# Autodesk Inventor assembly: Gantry Table With Chucks
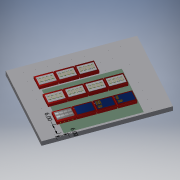
[picture p0: Inventor's stored thumbnail of the model, 180x180]
Saved by Autodesk Inventor 2019.4 (Build 234330000, 330)
## iProperties
Created: 2021-01-12
Part Number: Gantry Table With Chucks
Document SubType Name: Assembly
Designer: caleb
Author: caleb
## Documents named in this file (8)
- C:\Users\cfang\Desktop\nebraska-silicon-lab\Hardware\ETL\Module Assembly\Gantry Table With Chucks.iam
- C:\Users\cfang\Desktop\nebraska-silicon-lab\Hardware\ETL\Module Assembly\Gantry Base.ipt
- C:\Users\cfang\Desktop\nebraska-silicon-lab\Hardware\ETL\Module Assembly\Chuck with Assembly Plate.iam
- C:\Users\cfang\Desktop\nebraska-silicon-lab\Hardware\ETL\Module Assembly\Chuck with BBM Staging Plate.iam
- C:\Users\cfang\Desktop\nebraska-silicon-lab\Hardware\ETL\Module Assembly\Chuck with Glue Reservoir Plate.iam
- C:\Users\cfang\Desktop\nebraska-silicon-lab\Hardware\ETL\Module Assembly\Chuck with Glue Stamp Staging Plate.iam
- C:\Users\cfang\Desktop\nebraska-silicon-lab\Hardware\ETL\Module Assembly\Chuck\Chuck Assembly.iam
- C:\Users\cfang\Desktop\nebraska-silicon-lab\Hardware\ETL\Module Assembly\Glue Stamp Staging Plate\Assembly with Weights.iam
## Components (13 placed, 7 different names)
1. Gantry Base:1 — Mate:1, Mate:2, Mate:3, Mate:4, Angle:1, Angle:2, Angle:3, Angle:4, Mate:5, Angle:5, Mate:7, Mate:8, Mate:9, Angle:6, Angle:7, Angle:8, Mate:10, Mate:11, Mate:12, Angle:9, Angle:10, Angle:11, Insert:1, Insert:2, Insert:3, Insert:4, Insert:5, Insert:6, Insert:7, Insert:8, Insert:9, Insert:10, Insert:11
2. Chuck with Assembly Plate:1 [sub-assembly] — Mate:1, Angle:1, Insert:5
3. Chuck with BBM Staging Plate:1 [sub-assembly] — Mate:2, Angle:2, Insert:1
4. Chuck with Glue Reservoir Plate:1 [sub-assembly] — Mate:3, Angle:3, Insert:2
5. Chuck with Glue Stamp Staging Plate:1 [sub-assembly] — Mate:4, Angle:4, Insert:4
6. Chuck Assembly:1 [sub-assembly] — Mate:5, Angle:5, Mate:6, Tangent:1, Tangent:2, Tangent:3, Insert:3
7. Assembly with Weights:1 [sub-assembly] — Mate:6, Tangent:1, Tangent:2, Tangent:3
8. Chuck with Assembly Plate:2 [sub-assembly] — Mate:7, Angle:7, Insert:6
9. Chuck with Assembly Plate:3 [sub-assembly] — Mate:8, Angle:6, Insert:7
10. Chuck with Assembly Plate:4 [sub-assembly] — Mate:9, Angle:8, Insert:8
11. Chuck with Assembly Plate:5 [sub-assembly] — Mate:10, Angle:10, Insert:9
12. Chuck with Assembly Plate:6 [sub-assembly] — Mate:11, Angle:11, Insert:11
13. Chuck with Assembly Plate:7 [sub-assembly] — Mate:12, Angle:9, Insert:10
## Relationships (37: Mate 12, Angle 11, Insert 11, Tangent 3)
- Mate:1: Gantry Base:1 ↔ Chuck with Assembly Plate:1
- Mate:2: Gantry Base:1 ↔ Chuck with BBM Staging Plate:1
- Mate:3: Gantry Base:1 ↔ Chuck with Glue Reservoir Plate:1
- Mate:4: Gantry Base:1 ↔ Chuck with Glue Stamp Staging Plate:1
- Angle:1 (0 deg): Gantry Base:1 ↔ Chuck with Assembly Plate:1
- Angle:2 (0 deg): Gantry Base:1 ↔ Chuck with BBM Staging Plate:1
- Angle:3 (0 deg): Gantry Base:1 ↔ Chuck with Glue Reservoir Plate:1
- Angle:4 (0 deg): Gantry Base:1 ↔ Chuck with Glue Stamp Staging Plate:1
- Mate:5: Gantry Base:1 ↔ Chuck Assembly:1
- Angle:5 (0 deg): Gantry Base:1 ↔ Chuck Assembly:1
- Mate:6: Chuck Assembly:1 ↔ Assembly with Weights:1
- Tangent:1: Chuck Assembly:1 ↔ Assembly with Weights:1
- Tangent:2: Chuck Assembly:1 ↔ Assembly with Weights:1
- Tangent:3: Chuck Assembly:1 ↔ Assembly with Weights:1
- Mate:7: Gantry Base:1 ↔ Chuck with Assembly Plate:2
- Mate:8: Gantry Base:1 ↔ Chuck with Assembly Plate:3
- Mate:9: Gantry Base:1 ↔ Chuck with Assembly Plate:4
- Angle:6 (0 deg): Gantry Base:1 ↔ Chuck with Assembly Plate:3
- Angle:7 (0 deg): Gantry Base:1 ↔ Chuck with Assembly Plate:2
- Angle:8 (0 deg): Gantry Base:1 ↔ Chuck with Assembly Plate:4
- Mate:10: Gantry Base:1 ↔ Chuck with Assembly Plate:5
- Mate:11: Gantry Base:1 ↔ Chuck with Assembly Plate:6
- Mate:12: Gantry Base:1 ↔ Chuck with Assembly Plate:7
- Angle:9 (0 deg): Gantry Base:1 ↔ Chuck with Assembly Plate:7
- Angle:10 (0 deg): Gantry Base:1 ↔ Chuck with Assembly Plate:5
- Angle:11 (0 deg): Gantry Base:1 ↔ Chuck with Assembly Plate:6
- Insert:1: Gantry Base:1 ↔ Chuck with BBM Staging Plate:1
- Insert:2: Gantry Base:1 ↔ Chuck with Glue Reservoir Plate:1
- Insert:3: Gantry Base:1 ↔ Chuck Assembly:1
- Insert:4: Gantry Base:1 ↔ Chuck with Glue Stamp Staging Plate:1
- Insert:5: Gantry Base:1 ↔ Chuck with Assembly Plate:1
- Insert:6: Gantry Base:1 ↔ Chuck with Assembly Plate:2
- Insert:7: Gantry Base:1 ↔ Chuck with Assembly Plate:3
- Insert:8: Gantry Base:1 ↔ Chuck with Assembly Plate:4
- Insert:9: Gantry Base:1 ↔ Chuck with Assembly Plate:5
- Insert:10: Gantry Base:1 ↔ Chuck with Assembly Plate:7
- Insert:11: Gantry Base:1 ↔ Chuck with Assembly Plate:6
